# Autodesk Inventor assembly: Trucks
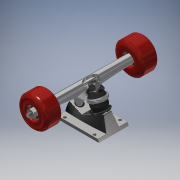
[picture p0: Inventor's stored thumbnail of the model, 180x180]
Saved by Autodesk Inventor 2019 (Build 230136000, 136)
## iProperties
Created: 2020-12-13
Part Number: Trucks
Document SubType Name: Assembly
Designer: Anass Hamdi
Author: Anass Hamdi
## Documents named in this file (11)
- C:\Users\Anass Hamdi\OneDrive - Vrije Universiteit Brussel\Documenten\Inventor\Anass Hamdi Project\Trucks.iam
- C:\Users\Anass Hamdi\OneDrive - Vrije Universiteit Brussel\Documenten\Inventor\Anass Hamdi Project\TruckBaseplate.iam
- C:\Users\Anass Hamdi\OneDrive - Vrije Universiteit Brussel\Documenten\Inventor\Anass Hamdi Project\UpperTruckPart.ipt
- C:\Users\Anass Hamdi\OneDrive - Vrije Universiteit Brussel\Documenten\Inventor\Anass Hamdi Project\BottomBushingWasherPart.ipt
- C:\Users\Anass Hamdi\OneDrive - Vrije Universiteit Brussel\Documenten\Inventor\Anass Hamdi Project\BushingBottomPart.ipt
- C:\Users\Anass Hamdi\OneDrive - Vrije Universiteit Brussel\Documenten\Inventor\Anass Hamdi Project\BushingTopPart.ipt
- C:\Users\Anass Hamdi\OneDrive - Vrije Universiteit Brussel\Documenten\Inventor\Anass Hamdi Project\TopBushingWasherPart.ipt
- C:\Users\Anass Hamdi\OneDrive - Vrije Universiteit Brussel\Documenten\Inventor\Anass Hamdi Project\KingPinNutPart.ipt
- C:\Users\Anass Hamdi\OneDrive - Vrije Universiteit Brussel\Documenten\Inventor\Anass Hamdi Project\WheelsWithBearings.iam
- C:\Users\Anass Hamdi\OneDrive - Vrije Universiteit Brussel\Documenten\Inventor\Anass Hamdi Project\AxleWasher.ipt
- C:\Users\Anass Hamdi\OneDrive - Vrije Universiteit Brussel\Documenten\Inventor\Anass Hamdi Project\AxleNut.ipt
## Components (15 placed, 10 different names)
1. TruckBaseplate:1 [sub-assembly] — Rigid:1, Rigid:2
2. UpperTruckPart:1 — Insert:1, Rigid:3, Rotational:5, Cylindrical:2, Rotational:8, Cylindrical:3
3. BottomBushingWasherPart:1 — Rigid:1
4. BushingBottomPart:1 — Rigid:2, Insert:1
5. BushingTopPart:1 — Rigid:3, Rigid:4
6. TopBushingWasherPart:1 — Rigid:4, Rigid:5
7. KingPinNutPart:1 — Rigid:5
8. WheelsWithBearings:2 [sub-assembly] — Rotational:4, Rotational:6
9. AxleWasher:1 — Rotational:4, Rotational:5
10. AxleWasher:2 — Rotational:6
11. AxleNut:2 — Cylindrical:2
12. WheelsWithBearings:3 [sub-assembly] — Rotational:7, Rotational:9
13. AxleNut:3 — Cylindrical:3
14. AxleWasher:3 — Rotational:9
15. AxleWasher:4 — Rotational:7, Rotational:8
## Relationships (14: RevoluteJoint 6, WeldJoint 5, CylindricalJoint 2, Insert 1)
- Rigid:1 [WeldJoint]: TruckBaseplate:1 ↔ BottomBushingWasherPart:1
- Rigid:2 [WeldJoint]: TruckBaseplate:1 ↔ BushingBottomPart:1
- Insert:1: UpperTruckPart:1 ↔ BushingBottomPart:1
- Rigid:3 [WeldJoint]: UpperTruckPart:1 ↔ BushingTopPart:1
- Rigid:4 [WeldJoint]: BushingTopPart:1 ↔ TopBushingWasherPart:1
- Rigid:5 [WeldJoint]: TopBushingWasherPart:1 ↔ KingPinNutPart:1
- Rotational:4 [RevoluteJoint]: WheelsWithBearings:2 ↔ AxleWasher:1
- Rotational:5 [RevoluteJoint]: UpperTruckPart:1 ↔ AxleWasher:1
- Rotational:6 [RevoluteJoint]: WheelsWithBearings:2 ↔ AxleWasher:2
- Cylindrical:2: UpperTruckPart:1 ↔ AxleNut:2
- Rotational:7 [RevoluteJoint]: WheelsWithBearings:3 ↔ AxleWasher:4
- Rotational:8 [RevoluteJoint]: UpperTruckPart:1 ↔ AxleWasher:4
- Rotational:9 [RevoluteJoint]: WheelsWithBearings:3 ↔ AxleWasher:3
- Cylindrical:3: UpperTruckPart:1 ↔ AxleNut:3
